# Autodesk Inventor assembly: Ensamble
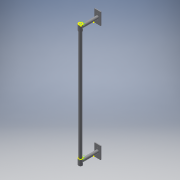
[picture p0: Inventor's stored thumbnail of the model, 180x180]
Saved by Autodesk Inventor 2018 (Build 220112000, 112)
## iProperties
Created: 2019-11-25
Part Number: Ensamble
Material: Genérico
Document SubType Name: Assembly
Designer: juanm
Author: juanm
## Documents named in this file (5)
- C:\Users\juanm\OneDrive\Documentos\Inventor\NombreProyecto\Ensamble.iam
- C:\Users\juanm\OneDrive\Documentos\Inventor\NombreProyecto\Soporte horizontal.ipt
- C:\Users\juanm\OneDrive\Documentos\Inventor\NombreProyecto\Soporte vertical.ipt
- C:\Users\juanm\OneDrive\Documentos\Inventor\NombreProyecto\Tornillo.ipt
- C:\Users\juanm\OneDrive\Documentos\Inventor\NombreProyecto\Pieza de unión.ipt
## Components (9 placed, 4 different names)
1. Soporte horizontal:1 — De rotación:1, De rotación:2
2. Soporte vertical:1 — De rotación:2, De rotación:5, De rotación:6, Rígido:2
3. Soporte vertical:2 — De rotación:1, De rotación:3, De rotación:4, Rígido:1
4. Tornillo:1 — De rotación:3
5. Tornillo:2 — De rotación:4
6. Tornillo:3 — De rotación:5
7. Tornillo:4 — De rotación:6
8. Pieza de unión:1 — Rígido:1
9. Pieza de unión:2 — Rígido:2
## Relationships (8: RevoluteJoint 6, WeldJoint 2)
- De rotación:1 [RevoluteJoint]: Soporte horizontal:1 ↔ Soporte vertical:2
- De rotación:2 [RevoluteJoint]: Soporte horizontal:1 ↔ Soporte vertical:1
- De rotación:3 [RevoluteJoint] (-25 mm): Soporte vertical:2 ↔ Tornillo:1
- De rotación:4 [RevoluteJoint] (-25 mm): Soporte vertical:2 ↔ Tornillo:2
- De rotación:5 [RevoluteJoint] (-25 mm): Soporte vertical:1 ↔ Tornillo:3
- De rotación:6 [RevoluteJoint] (-25 mm): Soporte vertical:1 ↔ Tornillo:4
- Rígido:1 [WeldJoint] (-135 mm): Soporte vertical:2 ↔ Pieza de unión:1
- Rígido:2 [WeldJoint] (-135 mm): Soporte vertical:1 ↔ Pieza de unión:2
